# Autodesk Inventor assembly: 0_Entire_Assembly
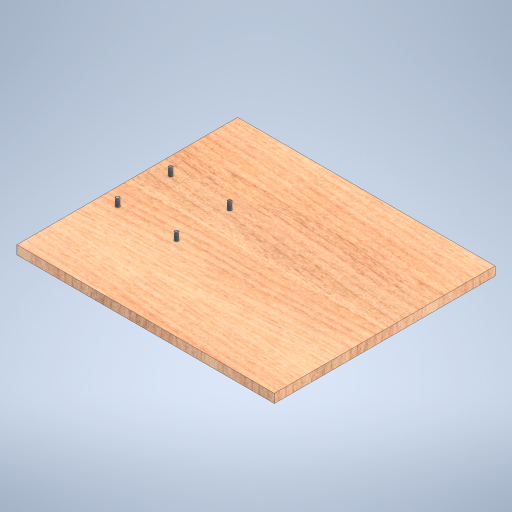
[picture p0: Inventor's stored thumbnail of the model, 512x512]
Saved by Autodesk Inventor 2024.2 (Build 282272000, 272)
## iProperties
Created: 2023-08-24
Part Number: 0_Entire_Assembly
Document SubType Name: Assembly
Designer: chanh
Author: chanh
## Documents named in this file (3)
- C:\Users\chanh\내 드라이브\로봇\Humanoid\Roboin Humanoid Project\Inventor\rh_plus_7_axis_robot_arm_hardware\Assembly\1_Base.iam
- C:\Users\chanh\내 드라이브\로봇\Humanoid\Roboin Humanoid Project\Inventor\rh_plus_7_axis_robot_arm_hardware\Part\Other Parts\base_plate.ipt
- C:\Users\chanh\내 드라이브\로봇\Humanoid\Roboin Humanoid Project\Inventor\rh_plus_7_axis_robot_arm_hardware\Part\Bolt, Bearing, Nut, Washer\M5x22 Flat Head Bolt.ipt
## Components (5 placed, 2 different names)
1. base_plate:1 — Flush:1, Flush:2, Flush:3, Rigid:1, Rigid:2, Rigid:3, Rigid:4
2. M5x22 Flat Head Bolt:1 — Rigid:3
3. M5x22 Flat Head Bolt:2 — Rigid:4
4. M5x22 Flat Head Bolt:3 — Rigid:1
5. M5x22 Flat Head Bolt:4 — Rigid:2
## Relationships (7: WeldJoint 4, Flush 3)
- Flush:1: base_plate:1
- Flush:2: base_plate:1
- Flush:3: base_plate:1
- Rigid:1 [WeldJoint]: base_plate:1 ↔ M5x22 Flat Head Bolt:3
- Rigid:2 [WeldJoint]: base_plate:1 ↔ M5x22 Flat Head Bolt:4
- Rigid:3 [WeldJoint]: base_plate:1 ↔ M5x22 Flat Head Bolt:1
- Rigid:4 [WeldJoint]: base_plate:1 ↔ M5x22 Flat Head Bolt:2
